# Autodesk Inventor assembly: Motor_MIR
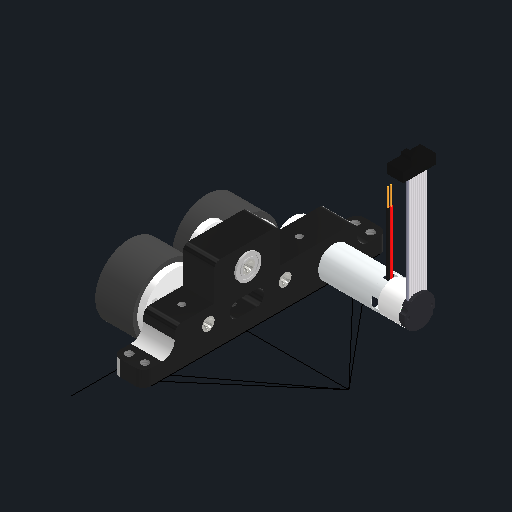
[picture p0: Inventor's stored thumbnail of the model, 512x512]
Saved by Autodesk Inventor 2022 (Build 260153000, 153)
## iProperties
Created: 2021-09-24
Part Number: Motor_MIR
Document SubType Name: Assembly
Designer: shiok
Author: shiok
## Documents named in this file (8)
- C:\Users\shiok\Documents\GitHub\murakumo\inventor\Motor_MIR.iam
- C:\Users\shiok\Documents\GitHub\murakumo\inventor\MotorBracket_MIR.ipt
- C:\Users\shiok\Documents\GitHub\murakumo\inventor\maxon DCX 10L_MIR.iam
- C:\Users\shiok\Documents\GitHub\murakumo\inventor\Tire_MIR.iam
- C:\Users\shiok\Documents\GitHub\murakumo\inventor\FL674ZZ_MIR.ipt
- C:\Users\shiok\Documents\GitHub\murakumo\inventor\shaft_short_MIR.ipt
- C:\Users\shiok\Documents\GitHub\murakumo\inventor\piniongear_41_middle_MIR.ipt
- C:\Users\shiok\Documents\GitHub\murakumo\inventor\piniongear_41_src_MIR.ipt
## Components (9 placed, 7 different names)
1. MotorBracket_MIR:1 — メイト:14, メイト:13, メイト:7, フラッシュ:4, フラッシュ:1, メイト:5, フラッシュ:3, メイト:6, フラッシュ:2, メイト:4, メイト:3, メイト:2, メイト:1
2. maxon DCX 10L_MIR:1 [sub-assembly] — メイト:14, メイト:13, メイト:7, メイト:12
3. Tire_MIR:1 [sub-assembly] — フラッシュ:4, フラッシュ:1, メイト:5, フラッシュ:7
4. Tire_MIR:2 [sub-assembly] — フラッシュ:3, メイト:6, フラッシュ:2
5. FL674ZZ_MIR:1 — メイト:4, メイト:3, メイト:10, フラッシュ:5
6. FL674ZZ_MIR:2 — メイト:2, メイト:1
7. shaft_short_MIR:1 — メイト:10, フラッシュ:5, フラッシュ:6, メイト:11
8. piniongear_41_middle_MIR:1 — フラッシュ:6, メイト:11
9. piniongear_41_src_MIR:1 — フラッシュ:7, メイト:12
## Relationships (19: Mate 12, Flush 7)
- メイト:14 [Mate]: MotorBracket_MIR:1 ↔ maxon DCX 10L_MIR:1
- メイト:13 [Mate]: MotorBracket_MIR:1 ↔ maxon DCX 10L_MIR:1
- メイト:7 [Mate]: MotorBracket_MIR:1 ↔ maxon DCX 10L_MIR:1
- フラッシュ:4 [Flush]: MotorBracket_MIR:1 ↔ Tire_MIR:1
- フラッシュ:1 [Flush]: MotorBracket_MIR:1 ↔ Tire_MIR:1
- メイト:5 [Mate]: MotorBracket_MIR:1 ↔ Tire_MIR:1
- フラッシュ:3 [Flush]: MotorBracket_MIR:1 ↔ Tire_MIR:2
- メイト:6 [Mate]: MotorBracket_MIR:1 ↔ Tire_MIR:2
- フラッシュ:2 [Flush]: MotorBracket_MIR:1 ↔ Tire_MIR:2
- メイト:4 [Mate]: MotorBracket_MIR:1 ↔ FL674ZZ_MIR:1
- メイト:3 [Mate]: MotorBracket_MIR:1 ↔ FL674ZZ_MIR:1
- メイト:2 [Mate]: MotorBracket_MIR:1 ↔ FL674ZZ_MIR:2
- メイト:1 [Mate]: MotorBracket_MIR:1 ↔ FL674ZZ_MIR:2
- メイト:10 [Mate]: FL674ZZ_MIR:1 ↔ shaft_short_MIR:1
- フラッシュ:5 [Flush]: FL674ZZ_MIR:1 ↔ shaft_short_MIR:1
- フラッシュ:6 [Flush]: shaft_short_MIR:1 ↔ piniongear_41_middle_MIR:1
- メイト:11 [Mate]: shaft_short_MIR:1 ↔ piniongear_41_middle_MIR:1
- フラッシュ:7 [Flush]: Tire_MIR:1 ↔ piniongear_41_src_MIR:1
- メイト:12 [Mate]: maxon DCX 10L_MIR:1 ↔ piniongear_41_src_MIR:1
